# Autodesk Inventor assembly: Assembly_full_final
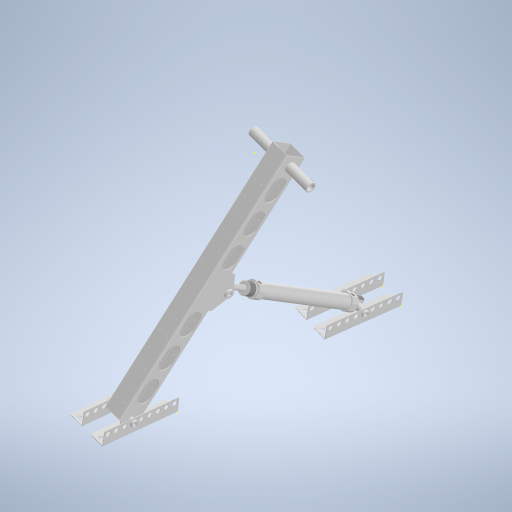
[picture p0: Inventor's stored thumbnail of the model, 512x512]
Saved by Autodesk Inventor 2023 (Build 270158000, 158)
## iProperties
Created: 2023-05-29
Part Number: Assembly_full_final
Document SubType Name: Assembly
Designer: steff
Author: steff
## Documents named in this file (16)
- C:\Users\steff\OneDrive\Skrivebord\uni\MER_MiniProject-main\3D Models\Assembly_full_final.iam
- C:\Users\steff\OneDrive\Skrivebord\uni\MER_MiniProject-main\3D Models\Base brackets\Mounting_bracket.ipt
- C:\Users\steff\OneDrive\Skrivebord\uni\MER_MiniProject-main\3D Models\Beam\BeamAssembly.iam
- C:\Users\steff\OneDrive\Skrivebord\uni\MER_MiniProject-main\3D Models\3D_print\CAD_A_Combined\CAD_A_inner.ipt
- C:\Users\steff\OneDrive\Skrivebord\uni\MER_MiniProject-main\3D Models\3D_print\CAD_A_Combined\CAD_A_outer v1.ipt
- C:\Users\steff\OneDrive\Skrivebord\uni\MER_MiniProject-main\3D Models\3D_print\CAD_A_Combined\CAD_A_outer_prop v1.ipt
- C:\Users\steff\OneDrive\Skrivebord\uni\MER_MiniProject-main\3D Models\3D_print\CAD_C_Combined\CAD_C_fill.ipt
- C:\Users\steff\OneDrive\Skrivebord\uni\MER_MiniProject-main\3D Models\3D_print\CAD_C_Combined\CAD_C_outer.ipt
- C:\Users\steff\OneDrive\Skrivebord\uni\MER_MiniProject-main\3D Models\3D_print\CAD_C_Combined\CAD_C_outer_prop.ipt
- C:\Users\steff\OneDrive\Skrivebord\uni\MER_MiniProject-main\3D Models\3D_print\CAD_C_Combined\CAD_inner_3.ipt
- C:\Users\steff\OneDrive\Skrivebord\uni\MER_MiniProject-main\3D Models\3D_print\CAD_B_Combined\CAD_B_inner v1.ipt
- C:\Users\steff\OneDrive\Skrivebord\uni\MER_MiniProject-main\3D Models\3D_print\CAD_B_Combined\CAD_B_inner_prop v1.ipt
- C:\Users\steff\OneDrive\Skrivebord\uni\MER_MiniProject-main\3D Models\3D_print\CAD_B_Combined\CAD_B_outer v1.ipt
- C:\Users\steff\OneDrive\Skrivebord\uni\MER_MiniProject-main\3D Models\3D_print\CAD_B_Combined\CAD_B_outer_prop v1.ipt
- C:\Users\steff\OneDrive\Skrivebord\uni\MER_MiniProject-main\3D Models\3D_print\CAD_B_Combined\CAD_B_fill.ipt
- C:\Users\steff\OneDrive\Skrivebord\uni\MER_MiniProject-main\3D Models\handle.ipt
## Components (27 placed, 15 different names)
1. Mounting_bracket:1 — Mate:45, Mate:46, Mate:50
2. Mounting_bracket:3 — Mate:41, Mate:42, Mate:47
3. BeamAssembly:1 [sub-assembly] — Mate:1, Mate:2, Mate:3, Mate:4, Mate:17, Mate:18, Mate:21, Mate:22, Mate:23, Mate:24, Mate:25, Mate:26, Mate:29, Mate:30, Mate:31, Mate:32, Mate:33, Mate:55, Mate:56, Flush:1
4. CAD_A_outer v1:1 — Mate:7, Mate:8, Mate:9, Mate:10, Mate:15
5. CAD_A_outer_prop v1:1 — Mate:15, Mate:16
6. CAD_A_outer v1:2 — Mate:5, Mate:6, Mate:51, Mate:52
7. CAD_A_inner:3 — Mate:1, Mate:2, Mate:5, Mate:6
8. CAD_A_inner:4 — Mate:3, Mate:4, Mate:7, Mate:8
9. Mounting_bracket:5 — Mate:9, Mate:10, Mate:16
10. CAD_C_fill:1 — Mate:27, Mate:28
11. CAD_C_outer:1 — Mate:29, Mate:30
12. CAD_inner_3:1 — Mate:17, Mate:18, Mate:19, Mate:20
13. CAD_C_outer:2 — Mate:21, Mate:22
14. CAD_C_outer_prop:2 — Mate:23, Mate:24
15. CAD_inner_3:3 — Mate:25, Mate:26, Mate:27, Mate:28
16. CAD_C_fill:3 — Mate:19, Mate:20
17. CAD_B_inner v1:1 — Mate:31, Mate:32, Mate:34, Mate:37, Mate:38
18. CAD_B_outer v1:1 — Mate:39, Mate:40, Mate:41, Mate:42, Mate:48
19. CAD_B_outer_prop v1:1 — Mate:49, Mate:50
20. CAD_B_inner_prop v1:2 — Mate:33, Mate:34, Mate:35, Mate:36
21. CAD_B_outer_prop v1:2 — Mate:47, Mate:48
22. CAD_B_fill:1 — Mate:35, Mate:36, Mate:43, Mate:44
23. CAD_B_fill:2 — Mate:37, Mate:38, Mate:39, Mate:40
24. CAD_B_outer v1:2 — Mate:43, Mate:44, Mate:45, Mate:46, Mate:49
25. CAD_A_outer_prop v1:4 — Mate:53, Mate:54
26. Mounting_bracket:7 — Mate:51, Mate:52, Mate:53, Mate:54
27. handle:1 — Mate:55, Mate:56, Flush:1
## Relationships (53: Mate 52, Flush 1)
- Mate:1: BeamAssembly:1 ↔ CAD_A_inner:3
- Mate:2: BeamAssembly:1 ↔ CAD_A_inner:3
- Mate:3: BeamAssembly:1 ↔ CAD_A_inner:4
- Mate:4: BeamAssembly:1 ↔ CAD_A_inner:4
- Mate:5: CAD_A_outer v1:2 ↔ CAD_A_inner:3
- Mate:6: CAD_A_outer v1:2 ↔ CAD_A_inner:3
- Mate:7: CAD_A_outer v1:1 ↔ CAD_A_inner:4
- Mate:8: CAD_A_outer v1:1 ↔ CAD_A_inner:4
- Mate:9: CAD_A_outer v1:1 ↔ Mounting_bracket:5
- Mate:10: CAD_A_outer v1:1 ↔ Mounting_bracket:5
- Mate:15: CAD_A_outer v1:1 ↔ CAD_A_outer_prop v1:1
- Mate:16: CAD_A_outer_prop v1:1 ↔ Mounting_bracket:5
- Mate:17: BeamAssembly:1 ↔ CAD_inner_3:1
- Mate:18: BeamAssembly:1 ↔ CAD_inner_3:1
- Mate:19: CAD_inner_3:1 ↔ CAD_C_fill:3
- Mate:20: CAD_inner_3:1 ↔ CAD_C_fill:3
- Mate:21: BeamAssembly:1 ↔ CAD_C_outer:2
- Mate:22: BeamAssembly:1 ↔ CAD_C_outer:2
- Mate:23: BeamAssembly:1 ↔ CAD_C_outer_prop:2
- Mate:24: BeamAssembly:1 ↔ CAD_C_outer_prop:2
- Mate:25: BeamAssembly:1 ↔ CAD_inner_3:3
- Mate:26: BeamAssembly:1 ↔ CAD_inner_3:3
- Mate:27: CAD_C_fill:1 ↔ CAD_inner_3:3
- Mate:28: CAD_C_fill:1 ↔ CAD_inner_3:3
- Mate:29: BeamAssembly:1 ↔ CAD_C_outer:1
- Mate:30: BeamAssembly:1 ↔ CAD_C_outer:1
- Mate:31: BeamAssembly:1 ↔ CAD_B_inner v1:1
- Mate:32: BeamAssembly:1 ↔ CAD_B_inner v1:1
- Mate:33: BeamAssembly:1 ↔ CAD_B_inner_prop v1:2
- Mate:34: CAD_B_inner v1:1 ↔ CAD_B_inner_prop v1:2
- Mate:35: CAD_B_inner_prop v1:2 ↔ CAD_B_fill:1
- Mate:36: CAD_B_inner_prop v1:2 ↔ CAD_B_fill:1
- Mate:37: CAD_B_inner v1:1 ↔ CAD_B_fill:2
- Mate:38: CAD_B_inner v1:1 ↔ CAD_B_fill:2
- Mate:39: CAD_B_outer v1:1 ↔ CAD_B_fill:2
- Mate:40: CAD_B_outer v1:1 ↔ CAD_B_fill:2
- Mate:41: Mounting_bracket:3 ↔ CAD_B_outer v1:1
- Mate:42: Mounting_bracket:3 ↔ CAD_B_outer v1:1
- Mate:43: CAD_B_fill:1 ↔ CAD_B_outer v1:2
- Mate:44: CAD_B_fill:1 ↔ CAD_B_outer v1:2
- Mate:45: Mounting_bracket:1 ↔ CAD_B_outer v1:2
- Mate:46: Mounting_bracket:1 ↔ CAD_B_outer v1:2
- Mate:47: Mounting_bracket:3 ↔ CAD_B_outer_prop v1:2
- Mate:48: CAD_B_outer v1:1 ↔ CAD_B_outer_prop v1:2
- Mate:49: CAD_B_outer_prop v1:1 ↔ CAD_B_outer v1:2
- Mate:50: Mounting_bracket:1 ↔ CAD_B_outer_prop v1:1
- Mate:51: CAD_A_outer v1:2 ↔ Mounting_bracket:7
- Mate:52: CAD_A_outer v1:2 ↔ Mounting_bracket:7
- Mate:53: CAD_A_outer_prop v1:4 ↔ Mounting_bracket:7
- Mate:54: CAD_A_outer_prop v1:4 ↔ Mounting_bracket:7
- Mate:55: BeamAssembly:1 ↔ handle:1
- Mate:56: BeamAssembly:1 ↔ handle:1
- Flush:1 (85 mm): BeamAssembly:1 ↔ handle:1
